# Autodesk Inventor assembly: STEFAN_2.0
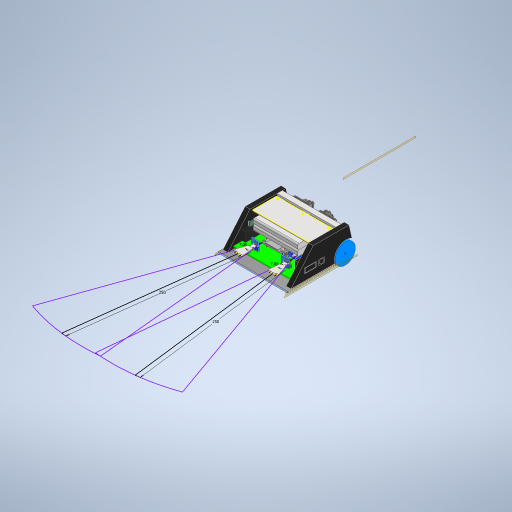
[picture p0: Inventor's stored thumbnail of the model, 512x512]
Saved by Autodesk Inventor 2023 (Build 270158000, 158)
## iProperties
Created: 2023-04-05
Part Number: STEFAN_2.0
Document SubType Name: Assembly
Designer: Kamil
Author: Kamil
## Documents named in this file (20)
- C:\Users\Kamil\Desktop\MojeRoboty\Stefan\mechanics\STEFAN_2.0.iam
- C:\Users\Kamil\Desktop\MojeRoboty\Stefan\mechanics\SCIANA_2.0.ipt
- C:\Users\Kamil\Desktop\MojeRoboty\Stefan\mechanics\n20 motor.ipt
- C:\Users\Kamil\Desktop\MojeRoboty\Stefan\mechanics\minisumopodsr.ipt
- C:\Users\Kamil\Desktop\MojeRoboty\Stefan\mechanics\uchwyt_na_silnik.ipt
- C:\Users\Kamil\Desktop\MojeRoboty\Stefan\mechanics\SCIANA_2.0_MIR.ipt
- C:\Users\Kamil\Desktop\MojeRoboty\Stefan\mechanics\PCB.ipt
- C:\Users\Kamil\Desktop\MojeRoboty\Stefan\mechanics\GP2Y0A41SK0F.ipt
- C:\Users\Kamil\Desktop\MojeRoboty\Stefan\mechanics\ESP32 v2.ipt
- C:\Users\Kamil\Desktop\MojeRoboty\Stefan\mechanics\motor drive module TB6612.ipt
- C:\Users\Kamil\Desktop\MojeRoboty\Stefan\mechanics\ARDUINO_NANO.ipt
- C:\Users\Kamil\Desktop\MojeRoboty\Stefan\mechanics\TOF_VLCOS.ipt
- C:\Users\Kamil\Desktop\MojeRoboty\Stefan\mechanics\GP2Y0A41SK0F_MIR1.ipt
- C:\Users\Kamil\Desktop\MojeRoboty\Stefan\mechanics\servo_stefan.ipt
- C:\Users\Kamil\Desktop\MojeRoboty\Stefan\mechanics\servo_stefan_MIR.ipt
- C:\Users\Kamil\Desktop\MojeRoboty\Stefan\mechanics\bateria szczurza.ipt
- C:\Users\Kamil\Desktop\MojeRoboty\Stefan\mechanics\opona_nowa.ipt
- C:\Users\Kamil\Desktop\MojeRoboty\Stefan\mechanics\mocowanie_serw.ipt
- C:\Users\Kamil\Desktop\MojeRoboty\Stefan\mechanics\PCBE_2_2.ipt
- C:\Users\Kamil\Desktop\MojeRoboty\Stefan\mechanics\pokrywka.ipt
## Components (23 placed, 19 different names)
1. SCIANA_2.0:1 — Zestawiające:7, Równoległe:6, Zestawiające:10, Równoległe:8, Zestawiające:11, Zestawiające:13, Równoległe:9, Zestawiające:20, Równoległe:15, Zestawiające:22, Równoległe:20, Równoległe:21, Równoległe:25
2. n20 motor:2 — Równoległe:4, Zestawiające:5, Równoległe:5, Zestawiające:6, Równoległe:19
3. minisumopodsr:1 — Równoległe:4, Zestawiające:1, Zestawiające:2, Zestawiające:3, Zestawiające:4, Zestawiające:7, Równoległe:6, Równoległe:7, Zestawiające:10, Równoległe:8
4. uchwyt_na_silnik:1 — Zestawiające:5, Równoległe:5, Zestawiające:6, Zestawiające:8, Zestawiające:9, Zestawiające:12
5. n20 motor:3 — Równoległe:7, Zestawiające:8, Zestawiające:9, Zestawiające:24
6. SCIANA_2.0_MIR:1 — Zestawiające:21
7. PCB:1 — Zestawiające:11, Zestawiające:12, Zestawiające:13, Zestawiające:14, Zestawiające:15, Zestawiające:16, Zestawiające:17, Równoległe:13, Równoległe:14
8. GP2Y0A41SK0F:1 — Równoległe:9, Zestawiające:14
9. ESP32 v2:1 — Zestawiające:15
10. motor drive module TB6612:1 — Zestawiające:16
11. ARDUINO_NANO:1 — Zestawiające:17
12. TOF_VLCOS:3 — Równoległe:13, Zestawiające:20
13. TOF_VLCOS:4 — Równoległe:14, Zestawiające:21
14. GP2Y0A41SK0F_MIR1:1
15. servo_stefan:1 — Równoległe:15, Zestawiające:22, Równoległe:16
16. servo_stefan_MIR:1 — Równoległe:16, Równoległe:23
17. bateria szczurza:1 — Zestawiające:23, Równoległe:17, Równoległe:18, Równoległe:21
18. bateria szczurza:2 — Zestawiające:23, Równoległe:17, Równoległe:18
19. opona_nowa:1 — Równoległe:19
20. opona_nowa:2 — Zestawiające:24, Równoległe:20
21. mocowanie_serw:1 — Równoległe:23, Równoległe:24
22. PCBE_2_2:1 — Równoległe:24
23. pokrywka:1 — Równoległe:25
## Relationships (41: Mate 22, Flush 18, Symmetry 1)
- Równoległe:4 [Flush]: n20 motor:2 ↔ minisumopodsr:1
- Zestawiające:1 [Mate]: minisumopodsr:1
- Zestawiające:2 [Mate]: minisumopodsr:1
- Zestawiające:3 [Mate]: minisumopodsr:1
- Zestawiające:4 [Mate]: minisumopodsr:1
- Symetria:1 [Symmetry]
- Zestawiające:5 [Mate]: n20 motor:2 ↔ uchwyt_na_silnik:1
- Równoległe:5 [Flush]: n20 motor:2 ↔ uchwyt_na_silnik:1
- Zestawiające:6 [Mate]: n20 motor:2 ↔ uchwyt_na_silnik:1
- Zestawiające:7 [Mate]: SCIANA_2.0:1 ↔ minisumopodsr:1
- Równoległe:6 [Flush] (1 mm): SCIANA_2.0:1 ↔ minisumopodsr:1
- Równoległe:7 [Flush]: minisumopodsr:1 ↔ n20 motor:3
- Zestawiające:8 [Mate]: uchwyt_na_silnik:1 ↔ n20 motor:3
- Zestawiające:9 [Mate]: uchwyt_na_silnik:1 ↔ n20 motor:3
- Zestawiające:10 [Mate]: SCIANA_2.0:1 ↔ minisumopodsr:1
- Równoległe:8 [Flush]: SCIANA_2.0:1 ↔ minisumopodsr:1
- Zestawiające:11 [Mate]: SCIANA_2.0:1 ↔ PCB:1
- Zestawiające:12 [Mate]: uchwyt_na_silnik:1 ↔ PCB:1
- Zestawiające:13 [Mate]: SCIANA_2.0:1 ↔ PCB:1
- Równoległe:9 [Flush]: SCIANA_2.0:1 ↔ GP2Y0A41SK0F:1
- Zestawiające:14 [Mate]: PCB:1 ↔ GP2Y0A41SK0F:1
- Zestawiające:15 [Mate] (8 mm): PCB:1 ↔ ESP32 v2:1
- Zestawiające:16 [Mate]: PCB:1 ↔ motor drive module TB6612:1
- Zestawiające:17 [Mate] (8 mm): PCB:1 ↔ ARDUINO_NANO:1
- Równoległe:13 [Flush]: PCB:1 ↔ TOF_VLCOS:3
- Równoległe:14 [Flush]: PCB:1 ↔ TOF_VLCOS:4
- Zestawiające:20 [Mate] (-25 mm): SCIANA_2.0:1 ↔ TOF_VLCOS:3
- Zestawiające:21 [Mate] (25 mm): SCIANA_2.0_MIR:1 ↔ TOF_VLCOS:4
- Równoległe:15 [Flush] (-3 mm): SCIANA_2.0:1 ↔ servo_stefan:1
- Zestawiające:22 [Mate] (7 mm): SCIANA_2.0:1 ↔ servo_stefan:1
- Równoległe:16 [Flush]: servo_stefan:1 ↔ servo_stefan_MIR:1
- Zestawiające:23 [Mate]: bateria szczurza:1 ↔ bateria szczurza:2
- Równoległe:17 [Flush]: bateria szczurza:1 ↔ bateria szczurza:2
- Równoległe:18 [Flush]: bateria szczurza:1 ↔ bateria szczurza:2
- Równoległe:19 [Flush]: n20 motor:2 ↔ opona_nowa:1
- Zestawiające:24 [Mate]: n20 motor:3 ↔ opona_nowa:2
- Równoległe:20 [Flush]: SCIANA_2.0:1 ↔ opona_nowa:2
- Równoległe:21 [Flush] (-3 mm): SCIANA_2.0:1 ↔ bateria szczurza:1
- Równoległe:23 [Flush]: servo_stefan_MIR:1 ↔ mocowanie_serw:1
- Równoległe:24 [Flush]: mocowanie_serw:1 ↔ PCBE_2_2:1
- Równoległe:25 [Flush]: SCIANA_2.0:1 ↔ pokrywka:1
